# Autodesk Inventor assembly: pvcconstruction
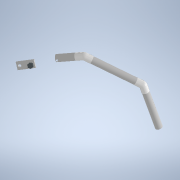
[picture p0: Inventor's stored thumbnail of the model, 180x180]
Saved by Autodesk Inventor 2021 (Build 250183000, 183)
## iProperties
Created: 2021-07-16
Part Number: pvcconstruction
Document SubType Name: Assembly
Designer: HP
Author: HP
## Documents named in this file (7)
- F:\Autodesk Invo\MII\pvcconstruction.iam
- F:\Autodesk Invo\MII\pvc up.ipt
- F:\Autodesk Invo\MII\45elbowfinal.ipt
- F:\Autodesk Invo\MII\PVC front 1.ipt
- F:\Autodesk Invo\MII\HOLDERPVC.ipt
- F:\Autodesk Invo\MII\holder.ipt
- F:\Autodesk Invo\MII\bolt.ipt
## Components (7 placed, 6 different names)
1. pvc up:1 — Mate:1, Mate:2, Mate:3, Mate:4
2. 45elbowfinal:1 — Mate:1, Mate:2, Mate:5, Mate:6
3. 45elbowfinal:2 — Mate:3, Mate:4, Mate:7, Mate:8
4. PVC front 1:1 — Mate:5, Mate:6
5. HOLDERPVC:1 — Mate:7, Mate:8
6. holder:1 — Cylindrical:1
7. bolt:1 — Cylindrical:1
## Relationships (9: Mate 8, CylindricalJoint 1)
- Mate:1: pvc up:1 ↔ 45elbowfinal:1
- Mate:2: pvc up:1 ↔ 45elbowfinal:1
- Mate:3: pvc up:1 ↔ 45elbowfinal:2
- Mate:4: pvc up:1 ↔ 45elbowfinal:2
- Mate:5: 45elbowfinal:1 ↔ PVC front 1:1
- Mate:6: 45elbowfinal:1 ↔ PVC front 1:1
- Mate:7: 45elbowfinal:2 ↔ HOLDERPVC:1
- Mate:8: 45elbowfinal:2 ↔ HOLDERPVC:1
- Cylindrical:1: holder:1 ↔ bolt:1
